# Autodesk Inventor assembly: Cajita
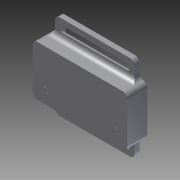
[picture p0: Inventor's stored thumbnail of the model, 180x180]
Saved by Autodesk Inventor 2012 (Build 160160000, 160)
## iProperties
Created: 2014-09-22
Part Number: Cajita
Document SubType Name: Assembly
Designer: SSepulveda
Author: SSepulveda
## Documents named in this file (3)
- C:\Users\SSepulveda\Documents\Cajita.iam
- C:\Users\SSepulveda\Documents\Part3.ipt
- C:\Users\SSepulveda\Documents\Part6.ipt
## Components (2 placed, 2 different names)
1. Base — Mate:1, Mate:2, Mate:3
2. Tapa — Mate:1, Mate:2, Mate:3
## Relationships (3: Mate 3)
- Mate:1: Base ↔ Tapa
- Mate:2: Base ↔ Tapa
- Mate:3: Base ↔ Tapa
